# Autodesk Inventor assembly: мёртвое колесо_MIR6_MIR_MIR1_MIR1
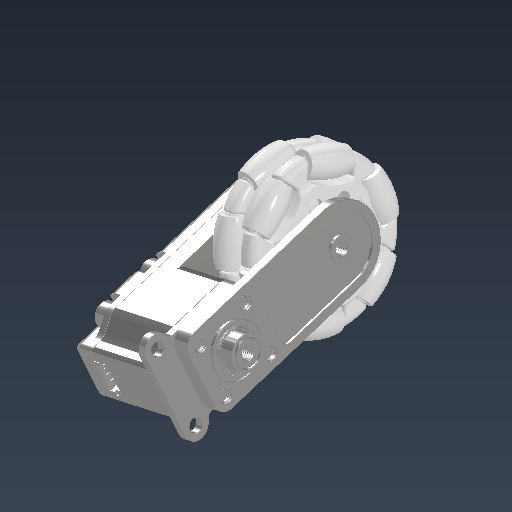
[picture p0: Inventor's stored thumbnail of the model, 512x512]
Saved by Autodesk Inventor 2026 (Build 300175000, 175)
## iProperties
Created: 2024-08-28
Part Number: мёртвое колесо_MIR6_MIR_MIR1_MIR1
Document SubType Name: Assembly
Designer: GameHD
Author: Phantom
## Documents named in this file (6)
- C:\Users\GameHD\Desktop\Phantom 16950\мёртвое колесо_MIR6_MIR_MIR1_MIR1.iam
- C:\Users\GameHD\Desktop\Phantom 16950\3110-0001-0001 assembly_MIR4_MIR_MIR1_MIR1.iam
- C:\Users\GameHD\Desktop\Phantom 16950\2915-0001-0003\2915-0001-0003_MIR2_MIR_MIR1_MIR1.ipt
- C:\Users\GameHD\Desktop\Phantom 16950\1502-0006-0120\1502-0006-0120_MIR2_MIR_MIR1_MIR1.ipt
- C:\Users\GameHD\Desktop\Phantom 16950\2800-0004-0020\2800-0004-0020_MIR2_MIR_MIR1_MIR1.ipt
- C:\Users\GameHD\Desktop\Phantom 16950\2812-0004-0007\2812-0004-0007_MIR2_MIR_MIR1_MIR1.ipt
## Components (5 placed, 5 different names)
1. 3110-0001-0001 assembly_MIR4_MIR_MIR1_MIR1:1 [sub-assembly]
2. 2915-0001-0003_MIR2_MIR_MIR1_MIR1:1 — Совмещение:5
3. 1502-0006-0120_MIR2_MIR_MIR1_MIR1:1 — Совмещение:4
4. 2800-0004-0020_MIR2_MIR_MIR1_MIR1:1 — Совмещение:5, Совмещение:4, Совмещение:5
5. 2812-0004-0007_MIR2_MIR_MIR1_MIR1:1 — Совмещение:5
## Relationships (3: Mate 3)
- Совмещение:5 [Mate]: 2915-0001-0003_MIR2_MIR_MIR1_MIR1:1 ↔ 2800-0004-0020_MIR2_MIR_MIR1_MIR1:1
- Совмещение:4 [Mate]: 1502-0006-0120_MIR2_MIR_MIR1_MIR1:1 ↔ 2800-0004-0020_MIR2_MIR_MIR1_MIR1:1
- Совмещение:5 [Mate]: 2800-0004-0020_MIR2_MIR_MIR1_MIR1:1 ↔ 2812-0004-0007_MIR2_MIR_MIR1_MIR1:1
